# Autodesk Inventor assembly: Assembly
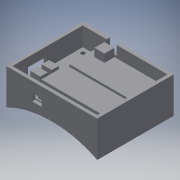
[picture p0: Inventor's stored thumbnail of the model, 180x180]
Saved by Autodesk Inventor 2017 (Build 210142000, 142)
## iProperties
Created: 2017-03-21
Part Number: Assembly
Document SubType Name: Assembly
Designer: Liam
Author: Liam
## Documents named in this file (4)
- C:\Users\Liam\Documents\GitHub\BiomedCapstone\Assembly.iam
- C:\Users\Liam\Documents\GitHub\BiomedCapstone\Base.ipt
- C:\Users\Liam\Documents\GitHub\BiomedCapstone\PCB.ipt
- C:\Users\Liam\Documents\GitHub\BiomedCapstone\Lid.ipt
## Components (3 placed, 3 different names)
1. Base:1 — Mate:1, Mate:2, Flush:1, Mate:3, Mate:4, Mate:5
2. PCB:1 — Mate:3, Mate:4, Mate:5
3. Lid:1 — Mate:1, Mate:2, Flush:1
## Relationships (6: Mate 5, Flush 1)
- Mate:1: Base:1 ↔ Lid:1
- Mate:2: Base:1 ↔ Lid:1
- Flush:1: Base:1 ↔ Lid:1
- Mate:3: Base:1 ↔ PCB:1
- Mate:4: Base:1 ↔ PCB:1
- Mate:5 (1 mm): Base:1 ↔ PCB:1
